# Autodesk Inventor assembly: sensor_board
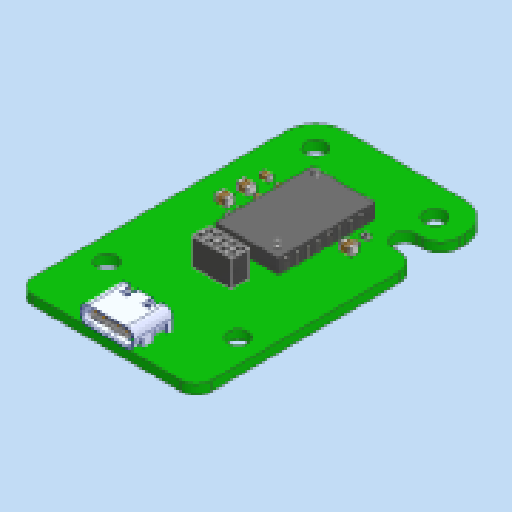
[picture p0: Inventor's stored thumbnail of the model, 512x512]
Saved by Autodesk Inventor 2024 (Build 280153000, 153)
## iProperties
Created: 2025-05-06
Part Number: sensor_board
Document SubType Name: Assembly
Designer: XxPan
Author: XxPan
## iProperties of the stored document CAP_0603.ipt
Created: 2025-05-07
Part Number: product
Material: Generic
Description: STEP AP214
Document SubType Name: Modeling
Designer: XxPan
Density: 1 g/cm^3
Appearance: Default
Title: CAP_CL10_SAM
Revision Number: 1.0first version
## iProperties of the stored document RES_0402.ipt
Created: 2025-05-06
Part Number: product
Material: Generic
Description: STEP AP214
Document SubType Name: Modeling
Designer: XxPan
Density: 1 g/cm^3
Appearance: Default
Title: RC0402N_YAG
Revision Number: 1.0first version
## iProperties of the stored document CAP_0805.ipt
Created: 2025-05-06
Part Number: product
Material: Generic
Description: STEP AP214
Document SubType Name: Modeling
Designer: XxPan
Density: 1 g/cm^3
Appearance: Default
Title: CAP_CL21_SAM
Revision Number: 1.0first version
## iProperties of the stored document CAP_0402.ipt
Created: 2025-05-06
Part Number: product
Material: Generic
Description: STEP AP214
Document SubType Name: Modeling
Designer: XxPan
Density: 1 g/cm^3
Appearance: Default
Title: CAP_CL05_SAM
Revision Number: 1.0first version
## iProperties of the stored document LPPB052CFFN-RC.ipt
Created: 2022-01-18
Part Number: LPPB052CFFN-RC
Material: Generic
Description: STEP AP214
Document SubType Name: Modeling
Designer: XxPan
Density: 1 g/cm^3
Appearance: Default
Sending System: SolidWorks 2020
Preprocessor: SwSTEP 2.0
Title: LPPB052CFFN-RC.STEP
Revision Number: ANY
## iProperties of the stored document 2171790001_2171790001.ipt
Created: 2025-05-10
Part Number: 2171790001_2171790001
Material: Generic
Document SubType Name: Modeling
Designer: XxPan
Density: 1 g/cm^3
Appearance: Default
Author: XxPan
Revision Number: ANY
## iProperties of the stored document 2171790001.iam
Created: 2023-11-14
Part Number: 2171790001
Description: STEP AP214
Document SubType Name: Assembly
Designer: XxPan
Sending System: SolidWorks 2021
Preprocessor: SwSTEP 2.0
Title: 2171790001.STEP
Revision Number: ANY
## Documents named in this file (17)
- C:\Users\XxPan\OneDrive - McMaster University\Mouse\CAD\sensor_board.iam
- C:\Users\XxPan\OneDrive - McMaster University\Mouse\CAD\PMW3360_sensor.ipt
- C:\Users\XxPan\OneDrive - McMaster University\Mouse\CAD\sensor_pcb.ipt
- **C:\Users\XxPan\OneDrive - McMaster University\Mouse\CAD\sensor_board.iam*LocalDocs*xAaaaaddaAaaaaaaaAaaaajjl1b*RES_0402.ipt
- **C:\Users\XxPan\OneDrive - McMaster University\Mouse\CAD\sensor_board.iam*LocalDocs*xAaaaaddaAaaaaaaaAaaaajjl4b*CAP_0603.ipt
- **C:\Users\XxPan\OneDrive - McMaster University\Mouse\CAD\sensor_board.iam*LocalDocs*xAaaaaddaAaaaaaaaAaaaajjlEc*CAP_0402.ipt
- **C:\Users\XxPan\OneDrive - McMaster University\Mouse\CAD\sensor_board.iam*LocalDocs*xAaaaaddaAaaaaaaaAaaaajjlIc*CAP_0805.ipt
- C:\Users\XxPan\OneDrive - McMaster University\Mouse\CAD\LM19-LSI_lens.ipt
- **C:\Users\XxPan\OneDrive - McMaster University\Mouse\CAD\sensor_board.iam*LocalDocs*xAaaaqtcaAaaaaaaaAaaaadrs4g*2171790001.iam
- **C:\Users\XxPan\OneDrive - McMaster University\Mouse\CAD\sensor_board.iam*LocalDocs*xAaaaqfcaAaaaaaaaAaaaq4rtNa*LPPB052CFFN-RC.ipt
- **C:\Users\XxPan\OneDrive - McMaster University\Mouse\CAD\sensor_board.iam*LocalDocs*xAaaaq3caAaaaaaaaAaaaahd5Jf*2171790001_2171790001.ipt
- C:\Users\XxPan\OneDrive - McMaster University\Mouse\CAD_models\resistors\RES_0402.step
- C:\Users\XxPan\OneDrive - McMaster University\Mouse\CAD_models\capacitors\CAP_0603.step
- C:\Users\XxPan\OneDrive - McMaster University\Mouse\CAD_models\capacitors\CAP_0402.step
- C:\Users\XxPan\OneDrive - McMaster University\Mouse\CAD_models\capacitors\CAP_0805.step
- C:\Users\XxPan\OneDrive - McMaster University\Mouse\CAD_models\2171790001 (USB-C, 16+8 dummy, SMD, board guide)\2171790001.step
- C:\Users\XxPan\OneDrive - McMaster University\Mouse\CAD_models\LPPB052CFFN_RC (2x5_P1.27mm_female_header)\LPPB052CFFN-RC.STEP
## Components (15 placed, 9 different names)
1. PMW3360_sensor:1 — Mate:1, Flush:6, Mate:23, Mate:24, Cylindrical:1, Angle:1, Mate:25
2. sensor_pcb:1 — Mate:1, Mate:8, Mate:9, Mate:10, Mate:11, Mate:12, Mate:13, Mate:14, Mate:15, Mate:16, Mate:17, Mate:21, Flush:1, Flush:2, Flush:3, Flush:4, Flush:5, Mate:22, Mate:25
3. RES_0402:1 — Mate:10
4. CAP_0603:1 — Mate:8
5. RES_0402:2 — Mate:9
6. CAP_0402:5 — Mate:12
7. CAP_0402:6 — Mate:15
8. CAP_0402:7 — Mate:14
9. CAP_0402:8 — Mate:16
10. CAP_0805:4 — Mate:17
11. CAP_0805:5 — Mate:13
12. CAP_0805:6 — Mate:11
13. LM19-LSI_lens:1 — Mate:24, Cylindrical:1, Angle:1
14. 2171790001:1 [sub-assembly] — Mate:21, Flush:2, Flush:5
15. LPPB052CFFN-RC:1 — Mate:22, Mate:23
## Relationships (24: Mate 16, Flush 6, CylindricalJoint 1, Angle 1)
- Mate:1: PMW3360_sensor:1 ↔ sensor_pcb:1
- Mate:8: sensor_pcb:1 ↔ CAP_0603:1
- Mate:9: sensor_pcb:1 ↔ RES_0402:2
- Mate:10: sensor_pcb:1 ↔ RES_0402:1
- Mate:11: sensor_pcb:1 ↔ CAP_0805:6
- Mate:12: sensor_pcb:1 ↔ CAP_0402:5
- Mate:13: sensor_pcb:1 ↔ CAP_0805:5
- Mate:14: sensor_pcb:1 ↔ CAP_0402:7
- Mate:15: sensor_pcb:1 ↔ CAP_0402:6
- Mate:16: sensor_pcb:1 ↔ CAP_0402:8
- Mate:17: sensor_pcb:1 ↔ CAP_0805:4
- Mate:21: sensor_pcb:1 ↔ 2171790001:1
- Flush:1: sensor_pcb:1
- Flush:2: sensor_pcb:1 ↔ 2171790001:1
- Flush:3: sensor_pcb:1
- Flush:4: sensor_pcb:1
- Flush:5: sensor_pcb:1 ↔ 2171790001:1
- Mate:22: sensor_pcb:1 ↔ LPPB052CFFN-RC:1
- Flush:6: PMW3360_sensor:1
- Mate:23 (3 mm): PMW3360_sensor:1 ↔ LPPB052CFFN-RC:1
- Mate:24 (-7.4 mm): PMW3360_sensor:1 ↔ LM19-LSI_lens:1
- Cylindrical:1: PMW3360_sensor:1 ↔ LM19-LSI_lens:1
- Angle:1 (0 deg): PMW3360_sensor:1 ↔ LM19-LSI_lens:1
- Mate:25: PMW3360_sensor:1 ↔ sensor_pcb:1
